# Autodesk Inventor assembly: SideCar5
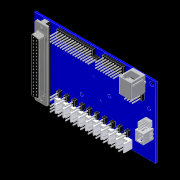
[picture p0: Inventor's stored thumbnail of the model, 180x180]
Saved by Autodesk Inventor 2012 (Build 160160000, 160)
## iProperties
Company: Team 801
Created: 2008-05-31
Part Number: SideCar5
Document SubType Name: Assembly
Designer: Jeffrey M
Catalog Web Link: www.team801.org
Mass: 26.5486 g
Surface Area: 344.727 cm^2
Volume: 26.5486 cm^3
Density: 1 g/cm^3
Translation Standard: STEP AP214IS
File Name: Open CASCADE Shape Model
Preprocessor: Open CASCADE 6.2
Postprocessor: Build: 320, Release: 2008 SP2 - Date: Mon 11/26/2007
Sent Units: MILLIMETERS
Uncertainty: 1e-06
Author: Jeffrey M
## Documents named in this file (11)
- Z:\UserData\Documents\Inventor\team1885frc\Electronics\DigitalSidecar\Sidecar Rev5 PCB Assembly.iam
- Z:\UserData\Documents\Inventor\team1885frc\Electronics\DigitalSidecar\HiTechnic_RJ_Plug.ipt
- Z:\UserData\Documents\Inventor\team1885frc\Electronics\DigitalSidecar\Sidecar Rev5 Board.ipt
- Z:\UserData\Documents\Inventor\team1885frc\Electronics\DigitalSidecar\Molex KK 2 Pin.ipt
- Z:\UserData\Documents\Inventor\team1885frc\Electronics\DigitalSidecar\Molex KK 3 Pin.ipt
- Z:\UserData\Documents\Inventor\team1885frc\Electronics\DigitalSidecar\Wago Power In.ipt
- Z:\UserData\Documents\Inventor\team1885frc\Electronics\DigitalSidecar\Jumper 2 Pin.ipt
- Z:\UserData\Documents\Inventor\team1885frc\Electronics\DigitalSidecar\DB37.ipt
- Z:\UserData\Documents\Inventor\team1885frc\Electronics\DigitalSidecar\J25.ipt
- Z:\UserData\Documents\Inventor\team1885frc\Electronics\DigitalSidecar\J21.ipt
- Z:\UserData\Documents\Inventor\team1885frc\Electronics\DigitalSidecar\J23.ipt
## Components (29 placed, 10 different names)
1. Sidecar Rev5 Board:1 — Mate:1, Mate:2, Mate:3, Mate:4, Mate:5, Mate:6, Mate:7, Mate:8, Mate:9, Mate:10, Mate:11, Mate:12, Mate:13, Mate:14, Mate:15, Mate:16, Mate:17, Mate:18, Flush:1, Mate:19, Tangent:1, Mate:20, Tangent:2, Mate:21, Tangent:3, Tangent:4
2. HiTechnic_RJ_Plug:1
3. Molex KK 2 Pin:1 — Mate:10, Mate:11, Mate:12
4. 734-132:1 — Mate:13, Mate:14, Mate:15
5. DB37:1 — Mate:1, Mate:2, Mate:3
6. Jumper 2 Pin:2 — Mate:16, Mate:17, Mate:18
7. J25:1 — Flush:1, Mate:19, Tangent:1, Flush:2
8. J21:1 — Mate:20, Flush:2, Tangent:2
9. J23:1 — Mate:21, Tangent:3, Tangent:4
10. Molex KK 3 Pin:1 — Mate:7, Mate:8, Mate:9
11. Jumper 2 Pin:1 — Mate:4, Mate:5, Mate:6
12. Molex KK 3 Pin:2
13. Jumper 2 Pin:3
14. Molex KK 3 Pin:3
15. Jumper 2 Pin:4
16. Molex KK 3 Pin:4
17. Jumper 2 Pin:5
18. Molex KK 3 Pin:5
19. Jumper 2 Pin:6
20. Molex KK 3 Pin:6
21. Jumper 2 Pin:7
22. Molex KK 3 Pin:7
23. Jumper 2 Pin:8
24. Molex KK 3 Pin:8
25. Jumper 2 Pin:9
26. Molex KK 3 Pin:9
27. Jumper 2 Pin:10
28. Molex KK 3 Pin:10
29. Jumper 2 Pin:11
## Component patterns: (10 elements, first: Molex KK 3 Pin:1 + Jumper 2 Pin:1)
## Relationships (27: Mate 21, Tangent 4, Flush 2)
- Mate:1: Sidecar Rev5 Board:1 ↔ DB37:1
- Mate:2: Sidecar Rev5 Board:1 ↔ DB37:1
- Mate:3: Sidecar Rev5 Board:1 ↔ DB37:1
- Mate:4: Sidecar Rev5 Board:1 ↔ Jumper 2 Pin:1
- Mate:5: Sidecar Rev5 Board:1 ↔ Jumper 2 Pin:1
- Mate:6: Sidecar Rev5 Board:1 ↔ Jumper 2 Pin:1
- Mate:7: Sidecar Rev5 Board:1 ↔ Molex KK 3 Pin:1
- Mate:8: Sidecar Rev5 Board:1 ↔ Molex KK 3 Pin:1
- Mate:9: Sidecar Rev5 Board:1 ↔ Molex KK 3 Pin:1
- Mate:10: Sidecar Rev5 Board:1 ↔ Molex KK 2 Pin:1
- Mate:11: Sidecar Rev5 Board:1 ↔ Molex KK 2 Pin:1
- Mate:12: Sidecar Rev5 Board:1 ↔ Molex KK 2 Pin:1
- Mate:13: Sidecar Rev5 Board:1 ↔ 734-132:1
- Mate:14: Sidecar Rev5 Board:1 ↔ 734-132:1
- Mate:15: Sidecar Rev5 Board:1 ↔ 734-132:1
- Mate:16: Sidecar Rev5 Board:1 ↔ Jumper 2 Pin:2
- Mate:17: Sidecar Rev5 Board:1 ↔ Jumper 2 Pin:2
- Mate:18: Sidecar Rev5 Board:1 ↔ Jumper 2 Pin:2
- Flush:1 (1.016 mm): Sidecar Rev5 Board:1 ↔ J25:1
- Mate:19: Sidecar Rev5 Board:1 ↔ J25:1
- Tangent:1 (-0.8255 mm): Sidecar Rev5 Board:1 ↔ J25:1
- Mate:20: Sidecar Rev5 Board:1 ↔ J21:1
- Flush:2: J25:1 ↔ J21:1
- Tangent:2 (-0.8255 mm): Sidecar Rev5 Board:1 ↔ J21:1
- Mate:21: Sidecar Rev5 Board:1 ↔ J23:1
- Tangent:3 (-0.8255 mm): Sidecar Rev5 Board:1 ↔ J23:1
- Tangent:4 (-0.8255 mm): Sidecar Rev5 Board:1 ↔ J23:1
